# Autodesk Inventor assembly: Motor
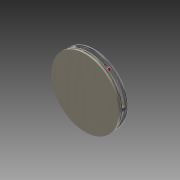
[picture p0: Inventor's stored thumbnail of the model, 180x180]
Saved by Autodesk Inventor 2014 (Build 180170000, 170)
## iProperties
Created: 2015-03-19
Part Number: Motor
Document SubType Name: Assembly
Designer: MSI
Author: MSI
## Documents named in this file (8)
- C:\Users\MSI\Dropbox\Ingenieursproject\inventor\Motor.iam
- C:\Users\MSI\Dropbox\Ingenieursproject\inventor\basis.ipt
- C:\Users\MSI\Dropbox\Ingenieursproject\inventor\lager.ipt
- C:\Users\MSI\Dropbox\Ingenieursproject\inventor\rotor.ipt
- C:\Users\MSI\Dropbox\Ingenieursproject\inventor\spoelhouder.ipt
- C:\Users\MSI\Dropbox\Ingenieursproject\inventor\Spoel.ipt
- C:\Users\MSI\Dropbox\Ingenieursproject\inventor\Kern.ipt
- C:\Users\MSI\Dropbox\Ingenieursproject\inventor\Hallhouder.ipt
## Components (18 placed, 7 different names)
1. basis:1 — Insert:1, Mate:1, Mate:2, Mate:3, Mate:4, Mate:5, Mate:6, Mate:7, Mate:8, Mate:9, Mate:10, Mate:11, Mate:12, Mate:13, Mate:14, Mate:15, Mate:16, Mate:17, Mate:18, Mate:25, Mate:26
2. lager:1 — Insert:1, Mate:19
3. rotor:1 — Mate:19, Mate:20
4. spoelhouder:1 — Mate:1, Mate:2, Mate:3, Insert:7
5. spoelhouder:2 — Mate:4, Mate:5, Mate:6, Insert:6
6. spoelhouder:3 — Mate:7, Mate:8, Mate:9, Insert:3
7. spoelhouder:4 — Mate:10, Mate:11, Mate:12, Insert:5
8. spoelhouder:5 — Mate:16, Mate:17, Mate:18, Insert:8
9. spoelhouder:6 — Mate:13, Mate:14, Mate:15, Insert:4
10. Spoel:1 — Insert:4
11. Spoel:2 — Insert:6, Mate:20, Mate:21
12. Spoel:3 — Insert:8, Mate:22
13. Spoel:4 — Insert:7, Mate:24
14. Spoel:5 — Insert:3, Mate:23
15. Spoel:6 — Insert:5
16. Kern:1 — Mate:21, Mate:22
17. Kern:2 — Mate:23, Mate:24
18. Hallhouder:1 — Mate:25, Mate:26
## Relationships (33: Mate 26, Insert 7)
- Insert:1: basis:1 ↔ lager:1
- Mate:1: basis:1 ↔ spoelhouder:1
- Mate:2: basis:1 ↔ spoelhouder:1
- Mate:3: basis:1 ↔ spoelhouder:1
- Mate:4: basis:1 ↔ spoelhouder:2
- Mate:5: basis:1 ↔ spoelhouder:2
- Mate:6: basis:1 ↔ spoelhouder:2
- Mate:7: basis:1 ↔ spoelhouder:3
- Mate:8: basis:1 ↔ spoelhouder:3
- Mate:9: basis:1 ↔ spoelhouder:3
- Mate:10: basis:1 ↔ spoelhouder:4
- Mate:11: basis:1 ↔ spoelhouder:4
- Mate:12: basis:1 ↔ spoelhouder:4
- Mate:13: basis:1 ↔ spoelhouder:6
- Mate:14: basis:1 ↔ spoelhouder:6
- Mate:15: basis:1 ↔ spoelhouder:6
- Mate:16: basis:1 ↔ spoelhouder:5
- Mate:17: basis:1 ↔ spoelhouder:5
- Mate:18: basis:1 ↔ spoelhouder:5
- Insert:3: spoelhouder:3 ↔ Spoel:5
- Insert:4: spoelhouder:6 ↔ Spoel:1
- Insert:5: spoelhouder:4 ↔ Spoel:6
- Insert:6: spoelhouder:2 ↔ Spoel:2
- Insert:7: spoelhouder:1 ↔ Spoel:4
- Insert:8: spoelhouder:5 ↔ Spoel:3
- Mate:19: lager:1 ↔ rotor:1
- Mate:20: rotor:1 ↔ Spoel:2
- Mate:21: Spoel:2 ↔ Kern:1
- Mate:22: Spoel:3 ↔ Kern:1
- Mate:23: Spoel:5 ↔ Kern:2
- Mate:24: Spoel:4 ↔ Kern:2
- Mate:25: basis:1 ↔ Hallhouder:1
- Mate:26: basis:1 ↔ Hallhouder:1
